# Autodesk Inventor assembly: assembly_fp15
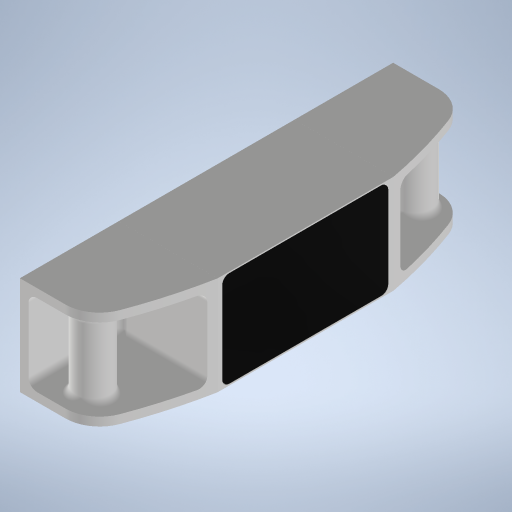
[picture p0: Inventor's stored thumbnail of the model, 512x512]
Saved by Autodesk Inventor 2023 (Build 270158000, 158)
## iProperties
Created: 2023-03-22
Part Number: assembly_fp15
Document SubType Name: Assembly
Designer: tdal0
Author: tdal0
## Documents named in this file (4)
- C:\4806\front panel parts\assembly_fp15.iam
- C:\4806\front panel parts\raspberry pi display.iam
- C:\4806\front panel parts\center_fp15.ipt
- C:\4806\front panel parts\sides_fp15.ipt
## Components (4 placed, 3 different names)
1. center_fp15:1 — Mate:1, Mate:2, Mate:3, Mate:4, Mate:5, Flush:1, Mate:6, Mate:7, Flush:2
2. raspberry pi display:1 [sub-assembly] — Mate:1, Mate:2, Mate:3
3. sides_fp15:1 — Mate:4, Mate:5, Flush:1
4. sides_fp15:2 — Mate:6, Mate:7, Flush:2
## Relationships (9: Mate 7, Flush 2)
- Mate:1: center_fp15:1 ↔ raspberry pi display:1
- Mate:2: center_fp15:1 ↔ raspberry pi display:1
- Mate:3: center_fp15:1 ↔ raspberry pi display:1
- Mate:4: center_fp15:1 ↔ sides_fp15:1
- Mate:5: center_fp15:1 ↔ sides_fp15:1
- Flush:1: center_fp15:1 ↔ sides_fp15:1
- Mate:6: center_fp15:1 ↔ sides_fp15:2
- Mate:7: center_fp15:1 ↔ sides_fp15:2
- Flush:2: center_fp15:1 ↔ sides_fp15:2
